# Autodesk Inventor assembly: Assembly2
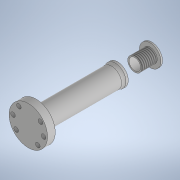
[picture p0: Inventor's stored thumbnail of the model, 180x180]
Saved by Autodesk Inventor 2022.2 (Build 262287000, 287)
## iProperties
Created: 2022-06-18
Part Number: Assembly2
Document SubType Name: Assembly
Designer: Usuario
Author: Usuario
## Documents named in this file (3)
- C:\Users\Usuario\OneDrive\Documentos\12\Robotics\Lab4\Assembly2.iam
- C:\Users\Usuario\OneDrive\Documentos\12\Robotics\Lab4\herramienta2.ipt
- C:\Users\Usuario\OneDrive\Documentos\12\Robotics\Lab4\Tapa.ipt
## Components (2 placed, 2 different names)
1. herramienta2:1 — Cylindrical:1
2. Tapa:1 — Cylindrical:1
## Relationships (1: CylindricalJoint 1)
- Cylindrical:1: herramienta2:1 ↔ Tapa:1
